# Autodesk Inventor assembly: 3A.03.JS.Wing test assembly
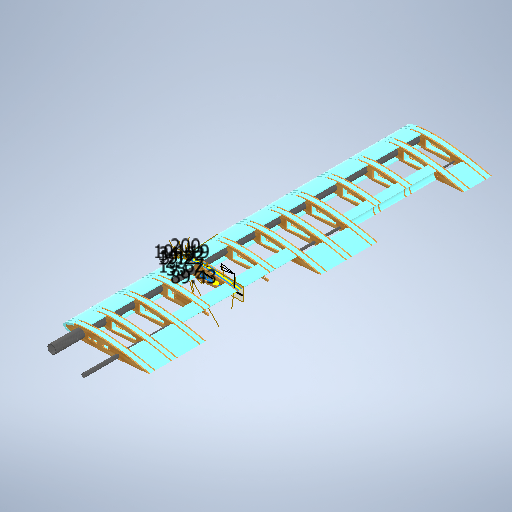
[picture p0: Inventor's stored thumbnail of the model, 512x512]
Saved by Autodesk Inventor 2025.1 (Build 291241000, 241)
## iProperties
Created: 2025-01-14
Part Number: 3A.03.JS.Wing test assembly
Document SubType Name: Assembly
Designer: johan
Author: johan
## Documents named in this file (30)
- C:\Users\johan\OneDrive - University of Bristol\CAD docs\2) Wing\3A.03.JS.Wing test assembly.iam
- C:\Users\johan\OneDrive - University of Bristol\CAD docs\2) Wing\2) Ribs\assemblies\3A.01.13.JS.Rib 13.iam
- C:\Users\johan\OneDrive - University of Bristol\CAD docs\2) Wing\3) Leading edge\assemblies\3A.04.01.JS.54mm root.iam
- C:\Users\johan\OneDrive - University of Bristol\CAD docs\2) Wing\2) Ribs\assemblies\3A.01.12.JS.Rib 12.iam
- C:\Users\johan\OneDrive - University of Bristol\CAD docs\2) Wing\3) Leading edge\assemblies\3A.04.02.JS.77mm.iam
- C:\Users\johan\OneDrive - University of Bristol\CAD docs\2) Wing\2) Ribs\assemblies\3A.01.11.JS.Rib 11.iam
- C:\Users\johan\OneDrive - University of Bristol\CAD docs\2) Wing\3) Leading edge\assemblies\3A.04.03.JS.74.75mm.iam
- C:\Users\johan\OneDrive - University of Bristol\CAD docs\2) Wing\3) Leading edge\assemblies\3A.04.04.90.75mm.iam
- C:\Users\johan\OneDrive - University of Bristol\CAD docs\2) Wing\2) Ribs\assemblies\3A.01.09.JS.Rib 9.iam
- C:\Users\johan\OneDrive - University of Bristol\CAD docs\2) Wing\2) Ribs\assemblies\3A.01.08.JS.Rib 8.iam
- C:\Users\johan\OneDrive - University of Bristol\CAD docs\2) Wing\2) Ribs\assemblies\3A.01.07.JS.Rib 7.iam
- C:\Users\johan\OneDrive - University of Bristol\CAD docs\2) Wing\3) Leading edge\assemblies\3A.04.05.JS.65.5mm.iam
- C:\Users\johan\OneDrive - University of Bristol\CAD docs\2) Wing\2) Ribs\assemblies\3A.01.06.JS.Rib 6.iam
- C:\Users\johan\OneDrive - University of Bristol\CAD docs\2) Wing\2) Ribs\assemblies\3A.01.05.JS.Rib 5.iam
- C:\Users\johan\OneDrive - University of Bristol\CAD docs\2) Wing\3) Leading edge\assemblies\3A.04.06.JS.84mm.iam
- C:\Users\johan\OneDrive - University of Bristol\CAD docs\2) Wing\2) Ribs\assemblies\3A.01.04.JS.Rib 4.iam
- C:\Users\johan\OneDrive - University of Bristol\CAD docs\2) Wing\2) Ribs\assemblies\3A.01.03.JS.Rib 3.iam
- C:\Users\johan\OneDrive - University of Bristol\CAD docs\2) Wing\2) Ribs\assemblies\3A.01.02.JS.Rib 2.iam
- C:\Users\johan\OneDrive - University of Bristol\CAD docs\2) Wing\3) Leading edge\assemblies\3A.04.07.JS.54mm tip.iam
- C:\Users\johan\OneDrive - University of Bristol\CAD docs\2) Wing\2) Ribs\assemblies\3A.01.01.JS.Rib 1.iam
- C:\Users\johan\OneDrive - University of Bristol\CAD docs\2) Wing\4) Trailing edge\3P.05.07.JS.flap trailing edge 90.ipt
- C:\Users\johan\OneDrive - University of Bristol\CAD docs\2) Wing\4) Trailing edge\3P.05.01.JS.trailing edge 54mm.ipt
- C:\Users\johan\OneDrive - University of Bristol\CAD docs\2) Wing\4) Trailing edge\3P.05.04JS.aileron trailing edge.ipt
- C:\Users\johan\OneDrive - University of Bristol\CAD docs\2) Wing\4) Trailing edge\3P.05.06.JS.flap trailing edge 74.ipt
- C:\Users\johan\OneDrive - University of Bristol\CAD docs\2) Wing\4) Trailing edge\3P.05.08.JS.trailing edge 65.5mm aileron.ipt
- C:\Users\johan\OneDrive - University of Bristol\CAD docs\2) Wing\4) Trailing edge\3P.05.09.JS.trailing edge 54mm aileron.ipt
- C:\Users\johan\OneDrive - University of Bristol\CAD docs\2) Wing\1) Spars\3P.01.GC.MAIN WING SPAR FINAL VERSION - updated.ipt
- C:\Users\johan\OneDrive - University of Bristol\CAD docs\2) Wing\4) Trailing edge\3P.05.02.JS.trailing edge 77mm.ipt
- C:\Users\johan\OneDrive - University of Bristol\CAD docs\2) Wing\1) Spars\Rear Wing Spar (tapered hollow).ipt
- C:\Users\johan\OneDrive - University of Bristol\CAD docs\2) Wing\2) Ribs\assemblies\3A.01.10.JS.Rib 10.iam
## Components (39 placed, 29 different names)
1. 3A.01.01.JS.Rib 1:1 [sub-assembly] — Rigid:24, Rigid:38, Rotational:1, Rotational:2
2. 3A.01.02.JS.Rib 2:1 [sub-assembly] — Rigid:22, Rigid:23
3. 3A.01.03.JS.Rib 3:1 [sub-assembly] — Rigid:20, Rigid:21, Rigid:34
4. 3A.01.04.JS.Rib 4:1 [sub-assembly] — Rigid:18, Rigid:19, Rigid:32, Rigid:33
5. 3A.01.05.JS.Rib 5:1 [sub-assembly] — Rigid:16, Rigid:17
6. 3A.01.06.JS.Rib 6:1 [sub-assembly] — Rigid:14, Rigid:15, Rigid:37
7. 3A.01.07.JS.Rib 7:1 [sub-assembly] — Rigid:12, Rigid:13, Rigid:40
8. 3A.01.08.JS.Rib 8:1 [sub-assembly] — Rigid:10, Rigid:11, Rigid:31
9. 3A.01.09.JS.Rib 9:1 [sub-assembly] — Rigid:8, Rigid:9, Rigid:29, Rigid:46
10. 3A.01.11.JS.Rib 11:1 [sub-assembly] — Rigid:4, Rigid:5
11. 3A.01.12.JS.Rib 12:1 [sub-assembly] — Rigid:2, Rigid:3, Rigid:39
12. 3A.01.13.JS.Rib 13:1 [sub-assembly] — Rigid:26, Rigid:27, Rigid:44
13. 3A.04.01.JS.54mm root:1 [sub-assembly] — Rigid:2, Rigid:27, Rigid:44
14. 3A.04.02.JS.77mm:1 [sub-assembly] — Rigid:3, Rigid:4
15. 3A.04.03.JS.74.75mm:1 [sub-assembly] — Rigid:5, Rigid:42
16. 3A.04.04.90.75mm:1 [sub-assembly] — Rigid:8, Rigid:41
17. 3A.04.05.JS.65.5mm:1 [sub-assembly] — Rigid:13, Rigid:14
18. 3A.04.06.JS.84mm:1 [sub-assembly] — Rigid:17, Rigid:18
19. 3A.04.07.JS.54mm tip:1 [sub-assembly] — Rigid:23, Rigid:24
20. 3A.04.04.90.75mm:2 [sub-assembly] — Rigid:9, Rigid:10
21. 3A.04.03.JS.74.75mm:2 [sub-assembly] — Rigid:11, Rigid:12
22. 3A.04.05.JS.65.5mm:2 [sub-assembly] — Rigid:15, Rigid:16
23. 3A.04.06.JS.84mm:2 [sub-assembly] — Rigid:19, Rigid:20
24. 3A.04.06.JS.84mm:3 [sub-assembly] — Rigid:21, Rigid:22
25. 3P.05.07.JS.flap trailing edge 90:1 — Rigid:46
26. 3P.05.01.JS.trailing edge 54mm:1 — Rigid:26
27. 3P.05.04JS.aileron trailing edge:1 — Rigid:32
28. 3P.05.06.JS.flap trailing edge 74:1 — Rigid:31
29. 3P.05.07.JS.flap trailing edge 90:2 — Rigid:29
30. 3P.05.06.JS.flap trailing edge 74:2 — Rigid:45
31. 3P.05.04JS.aileron trailing edge:2 — Rigid:34
32. 3P.05.04JS.aileron trailing edge:3 — Rigid:33
33. 3P.05.08.JS.trailing edge 65.5mm aileron:1 — Rigid:37
34. 3P.05.09.JS.trailing edge 54mm aileron:1 — Rigid:38
35. 3P.01.GC.MAIN WING SPAR FINAL VERSION - updated:1 — Rotational:1
36. 3P.05.02.JS.trailing edge 77mm:1 — Rigid:39
37. 3P.05.08.JS.trailing edge 65.5mm aileron:2 — Rigid:40
38. Rear Wing Spar (tapered hollow):1 — Rotational:2
39. 3A.01.10.JS.Rib 10:1 [sub-assembly] — Rigid:41, Rigid:42, Rigid:45
## Relationships (39: WeldJoint 37, RevoluteJoint 2)
- Rigid:2 [WeldJoint]: 3A.01.12.JS.Rib 12:1 ↔ 3A.04.01.JS.54mm root:1
- Rigid:3 [WeldJoint]: 3A.01.12.JS.Rib 12:1 ↔ 3A.04.02.JS.77mm:1
- Rigid:4 [WeldJoint]: 3A.01.11.JS.Rib 11:1 ↔ 3A.04.02.JS.77mm:1
- Rigid:5 [WeldJoint]: 3A.01.11.JS.Rib 11:1 ↔ 3A.04.03.JS.74.75mm:1
- Rigid:8 [WeldJoint]: 3A.01.09.JS.Rib 9:1 ↔ 3A.04.04.90.75mm:1
- Rigid:9 [WeldJoint]: 3A.01.09.JS.Rib 9:1 ↔ 3A.04.04.90.75mm:2
- Rigid:10 [WeldJoint]: 3A.01.08.JS.Rib 8:1 ↔ 3A.04.04.90.75mm:2
- Rigid:11 [WeldJoint]: 3A.01.08.JS.Rib 8:1 ↔ 3A.04.03.JS.74.75mm:2
- Rigid:12 [WeldJoint]: 3A.01.07.JS.Rib 7:1 ↔ 3A.04.03.JS.74.75mm:2
- Rigid:13 [WeldJoint]: 3A.01.07.JS.Rib 7:1 ↔ 3A.04.05.JS.65.5mm:1
- Rigid:14 [WeldJoint]: 3A.01.06.JS.Rib 6:1 ↔ 3A.04.05.JS.65.5mm:1
- Rigid:15 [WeldJoint]: 3A.01.06.JS.Rib 6:1 ↔ 3A.04.05.JS.65.5mm:2
- Rigid:16 [WeldJoint]: 3A.01.05.JS.Rib 5:1 ↔ 3A.04.05.JS.65.5mm:2
- Rigid:17 [WeldJoint]: 3A.01.05.JS.Rib 5:1 ↔ 3A.04.06.JS.84mm:1
- Rigid:18 [WeldJoint]: 3A.01.04.JS.Rib 4:1 ↔ 3A.04.06.JS.84mm:1
- Rigid:19 [WeldJoint]: 3A.01.04.JS.Rib 4:1 ↔ 3A.04.06.JS.84mm:2
- Rigid:20 [WeldJoint]: 3A.01.03.JS.Rib 3:1 ↔ 3A.04.06.JS.84mm:2
- Rigid:21 [WeldJoint]: 3A.01.03.JS.Rib 3:1 ↔ 3A.04.06.JS.84mm:3
- Rigid:22 [WeldJoint]: 3A.01.02.JS.Rib 2:1 ↔ 3A.04.06.JS.84mm:3
- Rigid:23 [WeldJoint]: 3A.01.02.JS.Rib 2:1 ↔ 3A.04.07.JS.54mm tip:1
- Rigid:24 [WeldJoint]: 3A.01.01.JS.Rib 1:1 ↔ 3A.04.07.JS.54mm tip:1
- Rigid:26 [WeldJoint]: 3A.01.13.JS.Rib 13:1 ↔ 3P.05.01.JS.trailing edge 54mm:1
- Rigid:27 [WeldJoint]: 3A.01.13.JS.Rib 13:1 ↔ 3A.04.01.JS.54mm root:1
- Rigid:29 [WeldJoint]: 3A.01.09.JS.Rib 9:1 ↔ 3P.05.07.JS.flap trailing edge 90:2
- Rigid:31 [WeldJoint]: 3A.01.08.JS.Rib 8:1 ↔ 3P.05.06.JS.flap trailing edge 74:1
- Rigid:32 [WeldJoint]: 3A.01.04.JS.Rib 4:1 ↔ 3P.05.04JS.aileron trailing edge:1
- Rigid:33 [WeldJoint]: 3A.01.04.JS.Rib 4:1 ↔ 3P.05.04JS.aileron trailing edge:3
- Rigid:34 [WeldJoint]: 3A.01.03.JS.Rib 3:1 ↔ 3P.05.04JS.aileron trailing edge:2
- Rigid:37 [WeldJoint]: 3A.01.06.JS.Rib 6:1 ↔ 3P.05.08.JS.trailing edge 65.5mm aileron:1
- Rigid:38 [WeldJoint]: 3A.01.01.JS.Rib 1:1 ↔ 3P.05.09.JS.trailing edge 54mm aileron:1
- Rigid:39 [WeldJoint]: 3A.01.12.JS.Rib 12:1 ↔ 3P.05.02.JS.trailing edge 77mm:1
- Rigid:40 [WeldJoint]: 3A.01.07.JS.Rib 7:1 ↔ 3P.05.08.JS.trailing edge 65.5mm aileron:2
- Rigid:41 [WeldJoint]: 3A.04.04.90.75mm:1 ↔ 3A.01.10.JS.Rib 10:1
- Rigid:42 [WeldJoint]: 3A.04.03.JS.74.75mm:1 ↔ 3A.01.10.JS.Rib 10:1
- Rigid:44 [WeldJoint]: 3A.01.13.JS.Rib 13:1 ↔ 3A.04.01.JS.54mm root:1
- Rigid:45 [WeldJoint]: 3P.05.06.JS.flap trailing edge 74:2 ↔ 3A.01.10.JS.Rib 10:1
- Rigid:46 [WeldJoint]: 3A.01.09.JS.Rib 9:1 ↔ 3P.05.07.JS.flap trailing edge 90:1
- Rotational:1 [RevoluteJoint]: 3A.01.01.JS.Rib 1:1 ↔ 3P.01.GC.MAIN WING SPAR FINAL VERSION - updated:1
- Rotational:2 [RevoluteJoint]: 3A.01.01.JS.Rib 1:1 ↔ Rear Wing Spar (tapered hollow):1
